# Autodesk Inventor assembly: PropellerAssembly
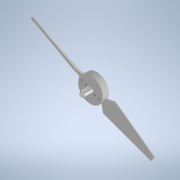
[picture p0: Inventor's stored thumbnail of the model, 180x180]
Saved by Autodesk Inventor 2021 (Build 250183000, 183)
## iProperties
Created: 2020-09-16
Part Number: PropellerAssembly
Document SubType Name: Assembly
Designer: Pysion
Mass: 19.7129 g
Surface Area: 140.019 cm^2
Volume: 19.7129 cm^3
Density: 1 g/cm^3
Author: Pysion
## Documents named in this file (7)
- C:\Users\Pysion\Documents\GrabCAD\V1\PropellerAssembly.iam
- C:\Users\Pysion\Documents\GrabCAD\V1\prop_base (1).ipt
- C:\Users\Pysion\Documents\GrabCAD\V1\prop_blade.ipt
- C:\Users\Pysion\Documents\GrabCAD\V1\prop_retaining_part.ipt
- C:\Users\Pysion\Documents\GrabCAD\V1\motor_shaft.ipt
- C:\Users\Pysion\Documents\GrabCAD\V1\ANSI B18.3 - 6-32 UNC - 0.4375(31).ipt
- C:\Users\Pysion\Documents\GrabCAD\V1\ANSI B18.3 - 6-32 UNC - 0.5(30).ipt
## Components (10 placed, 6 different names)
1. prop_base (1):1 — Mate:1, Mate:2, Angle:1, Mate:3, Mate:4, Flush:1, Mate:7, Mate:8, Flush:2, Mate:15, Mate:16, Mate:25, Mate:29
2. prop_blade:1 — Mate:1, Mate:2, Angle:1, Mate:19
3. prop_retaining_part:1 — Mate:3, Mate:4, Flush:1, Mate:20, Mate:21, Mate:22, Mate:24, Mate:26, Mate:27, Mate:28, Flush:3
4. motor_shaft:1 — Mate:7, Mate:8, Flush:2
5. prop_blade:2 — Mate:15, Mate:16, Angle:5, Mate:29
6. Hexagon Socket Flat Countersunk Head Cap Screw - Inch 6-32 UNC x 0.5:1 — Mate:28, Flush:3, Angle:6
7. Hexagon Socket Head Cap Screw - Inch No. 6 - 32 UNC - 7/16:4 — Mate:24, Mate:27, Angle:2, Angle:5
8. Hexagon Socket Head Cap Screw - Inch No. 6 - 32 UNC - 7/16:3 — Mate:25, Mate:26, Angle:2, Angle:3, Angle:6
9. Hexagon Socket Head Cap Screw - Inch No. 6 - 32 UNC - 7/16:1 — Mate:19, Mate:20, Angle:3, Angle:4
10. Hexagon Socket Head Cap Screw - Inch No. 6 - 32 UNC - 7/16:2 — Mate:21, Mate:22, Angle:4
## Relationships (27: Mate 18, Angle 6, Flush 3)
- Mate:1: prop_base (1):1 ↔ prop_blade:1
- Mate:2: prop_base (1):1 ↔ prop_blade:1
- Angle:1 (180 deg): prop_base (1):1 ↔ prop_blade:1
- Mate:3: prop_base (1):1 ↔ prop_retaining_part:1
- Mate:4: prop_base (1):1 ↔ prop_retaining_part:1
- Flush:1: prop_base (1):1 ↔ prop_retaining_part:1
- Mate:7 (0.05 mm): prop_base (1):1 ↔ motor_shaft:1
- Mate:8 (0.05 mm): prop_base (1):1 ↔ motor_shaft:1
- Flush:2: prop_base (1):1 ↔ motor_shaft:1
- Mate:15: prop_base (1):1 ↔ prop_blade:2
- Mate:16: prop_base (1):1 ↔ prop_blade:2
- Mate:19: prop_blade:1 ↔ Hexagon Socket Head Cap Screw - Inch No. 6 - 32 UNC - 7/16:1
- Mate:20: prop_retaining_part:1 ↔ Hexagon Socket Head Cap Screw - Inch No. 6 - 32 UNC - 7/16:1
- Mate:21: prop_retaining_part:1 ↔ Hexagon Socket Head Cap Screw - Inch No. 6 - 32 UNC - 7/16:2
- Mate:22: prop_retaining_part:1 ↔ Hexagon Socket Head Cap Screw - Inch No. 6 - 32 UNC - 7/16:2
- Mate:24: prop_retaining_part:1 ↔ Hexagon Socket Head Cap Screw - Inch No. 6 - 32 UNC - 7/16:4
- Mate:25: prop_base (1):1 ↔ Hexagon Socket Head Cap Screw - Inch No. 6 - 32 UNC - 7/16:3
- Mate:26: prop_retaining_part:1 ↔ Hexagon Socket Head Cap Screw - Inch No. 6 - 32 UNC - 7/16:3
- Mate:27: prop_retaining_part:1 ↔ Hexagon Socket Head Cap Screw - Inch No. 6 - 32 UNC - 7/16:4
- Mate:28: prop_retaining_part:1 ↔ Hexagon Socket Flat Countersunk Head Cap Screw - Inch 6-32 UNC x 0.5:1
- Flush:3: prop_retaining_part:1 ↔ Hexagon Socket Flat Countersunk Head Cap Screw - Inch 6-32 UNC x 0.5:1
- Angle:2 (0 deg): Hexagon Socket Head Cap Screw - Inch No. 6 - 32 UNC - 7/16:4 ↔ Hexagon Socket Head Cap Screw - Inch No. 6 - 32 UNC - 7/16:3
- Angle:3 (0 deg): Hexagon Socket Head Cap Screw - Inch No. 6 - 32 UNC - 7/16:3 ↔ Hexagon Socket Head Cap Screw - Inch No. 6 - 32 UNC - 7/16:1
- Angle:4 (0 deg): Hexagon Socket Head Cap Screw - Inch No. 6 - 32 UNC - 7/16:1 ↔ Hexagon Socket Head Cap Screw - Inch No. 6 - 32 UNC - 7/16:2
- Angle:5 (0 deg): prop_blade:2 ↔ Hexagon Socket Head Cap Screw - Inch No. 6 - 32 UNC - 7/16:4
- Mate:29: prop_base (1):1 ↔ prop_blade:2
- Angle:6 (0 deg): Hexagon Socket Flat Countersunk Head Cap Screw - Inch 6-32 UNC x 0.5:1 ↔ Hexagon Socket Head Cap Screw - Inch No. 6 - 32 UNC - 7/16:3
